# Autodesk Inventor assembly: pallet_step_with_pipe
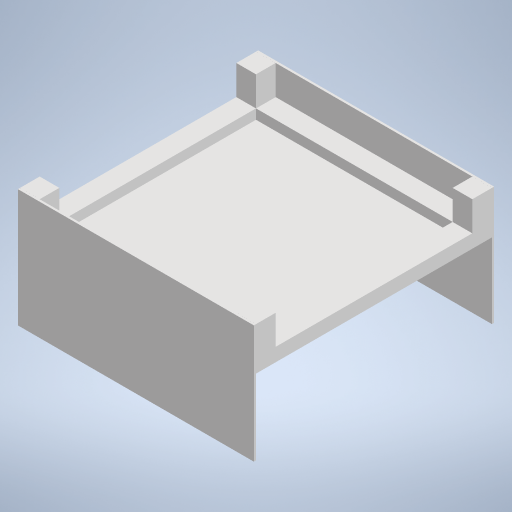
[picture p0: Inventor's stored thumbnail of the model, 512x512]
Saved by Autodesk Inventor 2024 (Build 280153000, 153)
## iProperties
Created: 2024-01-12
Part Number: pallet_step_with_pipe
Document SubType Name: Assembly
Designer: nicky
Author: nicky
## Documents named in this file (5)
- D:\OneDrive - 성균관대학교\Projects\2024 ICRA QRC 대회\모델\pallet_step_with_pipe.iam
- D:\OneDrive - 성균관대학교\Projects\2024 ICRA QRC 대회\모델\pallet_step.iam
- D:\OneDrive - 성균관대학교\Projects\2024 ICRA QRC 대회\모델\board_50x100x1200.ipt
- D:\OneDrive - 성균관대학교\Projects\2024 ICRA QRC 대회\모델\board_50x100x300.ipt
- D:\OneDrive - 성균관대학교\Projects\2024 ICRA QRC 대회\모델\board_11x600x1200.ipt
## Components (6 placed, 4 different names)
1. pallet_step:1 [sub-assembly] — 플러쉬:1, 메이트:1, 플러쉬:2, 플러쉬:3, 메이트:2, 플러쉬:4, 플러쉬:5, 플러쉬:6, 플러쉬:7
2. board_50x100x1200:1 — 플러쉬:1, 메이트:1, 플러쉬:2, 메이트:3
3. board_50x100x300:1 — 플러쉬:3, 메이트:4
4. board_50x100x300:2 — 메이트:2, 플러쉬:4, 메이트:3
5. board_11x600x1200:1 — 플러쉬:5
6. board_11x600x1200:2 — 메이트:4, 플러쉬:6, 플러쉬:7
## Relationships (11: Flush 7, Mate 4)
- 플러쉬:1 [Flush]: pallet_step:1 ↔ board_50x100x1200:1
- 메이트:1 [Mate]: pallet_step:1 ↔ board_50x100x1200:1
- 플러쉬:2 [Flush]: pallet_step:1 ↔ board_50x100x1200:1
- 플러쉬:3 [Flush]: pallet_step:1 ↔ board_50x100x300:1
- 메이트:2 [Mate]: pallet_step:1 ↔ board_50x100x300:2
- 플러쉬:4 [Flush]: pallet_step:1 ↔ board_50x100x300:2
- 메이트:3 [Mate]: board_50x100x1200:1 ↔ board_50x100x300:2
- 플러쉬:5 [Flush]: pallet_step:1 ↔ board_11x600x1200:1
- 메이트:4 [Mate]: board_50x100x300:1 ↔ board_11x600x1200:2
- 플러쉬:6 [Flush]: pallet_step:1 ↔ board_11x600x1200:2
- 플러쉬:7 [Flush]: pallet_step:1 ↔ board_11x600x1200:2
